# Autodesk Inventor assembly: EnclosureAssembly
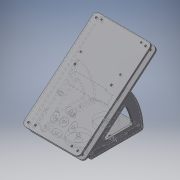
[picture p0: Inventor's stored thumbnail of the model, 180x180]
Saved by Autodesk Inventor 2016 (Build 200138000, 138)
## iProperties
Created: 2016-07-10
Part Number: EnclosureAssembly
Document SubType Name: Assembly
Designer: jeffkub
Author: jeffkub
## Documents named in this file (6)
- E:\Projects\beer-gauge\enclosure\EnclosureAssembly.iam
- E:\Projects\beer-gauge\enclosure\MountBase.ipt
- E:\Projects\beer-gauge\enclosure\SideMount.ipt
- E:\Projects\beer-gauge\enclosure\BackCover.ipt
- E:\Projects\beer-gauge\enclosure\FrontCover.ipt
- E:\Projects\beer-gauge\enclosure\Magnet.ipt
## Components (7 placed, 5 different names)
1. MountBase:1 — Flush:1, Flush:2, Flush:3, Mate:1, Mate:2, Mate:3, Mate:4, Mate:5, Mate:6, Mate:12, Mate:13, Mate:14, Mate:15
2. SideMount:1 — Mate:1, Mate:2, Mate:3, Mate:7
3. SideMount:2 — Mate:4, Mate:5, Mate:6, Mate:8, Mate:9
4. BackCover:1 — Mate:7, Mate:8, Mate:9, Mate:10, Flush:4, Mate:11
5. FrontCover:1 — Mate:10, Flush:4, Mate:11
6. Magnet:1 — Mate:12, Mate:13
7. Magnet:2 — Mate:14, Mate:15
## Relationships (19: Mate 15, Flush 4)
- Flush:1: MountBase:1
- Flush:2: MountBase:1
- Flush:3: MountBase:1
- Mate:1: MountBase:1 ↔ SideMount:1
- Mate:2: MountBase:1 ↔ SideMount:1
- Mate:3 (-0.1 mm): MountBase:1 ↔ SideMount:1
- Mate:4: MountBase:1 ↔ SideMount:2
- Mate:5: MountBase:1 ↔ SideMount:2
- Mate:6 (-0.1 mm): MountBase:1 ↔ SideMount:2
- Mate:7 (-0.1 mm): SideMount:1 ↔ BackCover:1
- Mate:8: SideMount:2 ↔ BackCover:1
- Mate:9: SideMount:2 ↔ BackCover:1
- Mate:10 (10 mm): BackCover:1 ↔ FrontCover:1
- Flush:4: BackCover:1 ↔ FrontCover:1
- Mate:11: BackCover:1 ↔ FrontCover:1
- Mate:12: MountBase:1 ↔ Magnet:1
- Mate:13: MountBase:1 ↔ Magnet:1
- Mate:14: MountBase:1 ↔ Magnet:2
- Mate:15: MountBase:1 ↔ Magnet:2
